# Autodesk Inventor assembly: Enclosure Assembly
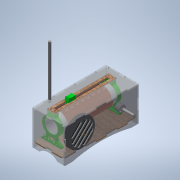
[picture p0: Inventor's stored thumbnail of the model, 180x180]
Saved by Autodesk Inventor 2021 (Build 250183000, 183)
## iProperties
Created: 2017-12-06
Part Number: Enclosure Assembly
Document SubType Name: Assembly
Designer: Andrew
Author: Andrew
## Documents named in this file (11)
- D:\OneDrive\3D Models\AM Radio\Enclosure Assembly.iam
- D:\OneDrive\3D Models\AM Radio\Knob Assembly.iam
- D:\OneDrive\3D Models\AM Radio\Potentiometer.ipt
- D:\OneDrive\3D Models\AM Radio\Enclosure Front.ipt
- D:\OneDrive\3D Models\AM Radio\Enclosure Top.ipt
- D:\OneDrive\3D Models\AM Radio\Enclosure Back.ipt
- D:\OneDrive\3D Models\AM Radio\Speaker.ipt
- D:\OneDrive\3D Models\AM Radio\Enclosure Side.ipt
- D:\OneDrive\3D Models\AM Radio\Enclosure Bottom.ipt
- D:\OneDrive\3D Models\AM Radio\Inductor Assembly.iam
- D:\OneDrive\3D Models\AM Radio\Antenna.ipt
## Components (11 placed, 10 different names)
1. Knob Assembly:1 [sub-assembly] — Mate:1, Mate:2
2. Potentiometer:1 — Mate:1, Mate:2, Mate:3, Mate:4
3. Enclosure Front:1 — Flush:1, Flush:2, Flush:3, Mate:3, Mate:4, Mate:5, Flush:5, Flush:6, Flush:12, Flush:13, Flush:14, Flush:15, Mate:11, Mate:12, Mate:13
4. Enclosure Top:1 — Flush:4, Mate:5, Flush:5, Flush:6, Flush:8, Flush:10, Flush:11, Mate:8, Mate:9, Flush:16, Flush:17, Flush:19, Mate:14, Mate:15, Mate:16
5. Enclosure Back:1 — Flush:8, Flush:18, Flush:19
6. Speaker:1 — Mate:11, Mate:12
7. Enclosure Side:1 — Flush:11, Flush:13, Flush:15
8. Enclosure Side:2 — Flush:10, Flush:12, Flush:14, Flush:18
9. Enclosure Bottom:1 — Flush:16, Flush:17, Mate:13
10. Inductor Assembly:1 [sub-assembly] — Mate:8, Mate:9
11. Antenna:1 — Mate:14, Mate:15, Mate:16
## Relationships (30: Flush 17, Mate 13)
- Mate:1: Knob Assembly:1 ↔ Potentiometer:1
- Mate:2: Knob Assembly:1 ↔ Potentiometer:1
- Flush:1: Enclosure Front:1
- Flush:2: Enclosure Front:1
- Flush:3: Enclosure Front:1
- Mate:3: Potentiometer:1 ↔ Enclosure Front:1
- Mate:4: Potentiometer:1 ↔ Enclosure Front:1
- Flush:4: Enclosure Top:1
- Mate:5: Enclosure Front:1 ↔ Enclosure Top:1
- Flush:5: Enclosure Front:1 ↔ Enclosure Top:1
- Flush:6: Enclosure Front:1 ↔ Enclosure Top:1
- Flush:8: Enclosure Top:1 ↔ Enclosure Back:1
- Flush:10: Enclosure Top:1 ↔ Enclosure Side:2
- Flush:11: Enclosure Top:1 ↔ Enclosure Side:1
- Flush:12: Enclosure Front:1 ↔ Enclosure Side:2
- Flush:13: Enclosure Front:1 ↔ Enclosure Side:1
- Flush:14: Enclosure Front:1 ↔ Enclosure Side:2
- Flush:15: Enclosure Front:1 ↔ Enclosure Side:1
- Mate:8 (0.635 mm): Enclosure Top:1 ↔ Inductor Assembly:1
- Mate:9 (0.635 mm): Enclosure Top:1 ↔ Inductor Assembly:1
- Flush:16: Enclosure Top:1 ↔ Enclosure Bottom:1
- Flush:17: Enclosure Top:1 ↔ Enclosure Bottom:1
- Mate:11: Enclosure Front:1 ↔ Speaker:1
- Mate:12: Enclosure Front:1 ↔ Speaker:1
- Mate:13 (0.35 mm): Enclosure Front:1 ↔ Enclosure Bottom:1
- Flush:18: Enclosure Back:1 ↔ Enclosure Side:2
- Flush:19: Enclosure Top:1 ↔ Enclosure Back:1
- Mate:14: Enclosure Top:1 ↔ Antenna:1
- Mate:15: Enclosure Top:1 ↔ Antenna:1
- Mate:16: Enclosure Top:1 ↔ Antenna:1
